# Autodesk Inventor assembly: Carril
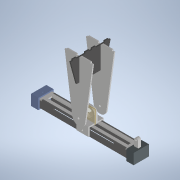
[picture p0: Inventor's stored thumbnail of the model, 180x180]
Saved by Autodesk Inventor 2022 (Build 260153000, 153)
## iProperties
Created: 2022-01-30
Part Number: Carril
Document SubType Name: Assembly
Designer: katha
Author: katha
## Documents named in this file (8)
- C:\Users\katha\OneDrive\Escritorio\Mini_Proyecto_Diseno\Diseno_18012\Modelo_MPD\Carril.iam
- C:\Users\katha\OneDrive\Escritorio\Mini_Proyecto_Diseno\Diseno_18012\Modelo_MPD\Lateral_Carril.ipt
- C:\Users\katha\OneDrive\Escritorio\Mini_Proyecto_Diseno\Diseno_18012\Modelo_MPD\Base_Carril.ipt
- C:\Users\katha\OneDrive\Escritorio\Mini_Proyecto_Diseno\Diseno_18012\Modelo_MPD\Tope_Carril.ipt
- C:\Users\katha\OneDrive\Escritorio\Mini_Proyecto_Diseno\Diseno_18012\Modelo_MPD\Tope_Carril_derecho.ipt
- C:\Users\katha\OneDrive\Escritorio\Mini_Proyecto_Diseno\Diseno_18012\Modelo_MPD\Eje_Carril.ipt
- C:\Users\katha\OneDrive\Escritorio\Mini_Proyecto_Diseno\Diseno_18012\Modelo_MPD\Base.ipt
- C:\Users\katha\OneDrive\Escritorio\Mini_Proyecto_Diseno\Diseno_18012\Modelo_MPD\Base_Soporte.ipt
## Components (9 placed, 7 different names)
1. Lateral_Carril:1 — Flush:1, Flush:3, Mate:2, Mate:4, Mate:7, Mate:18
2. Lateral_Carril:2 — Flush:2, Flush:4, Mate:1, Mate:10
3. Base_Carril:1 — Flush:1, Flush:2, Flush:3, Flush:4, Mate:1, Mate:2, Mate:3, Mate:5, Mate:6, Mate:8, Mate:17
4. Tope_Carril:1 — Mate:3, Mate:4, Mate:5
5. Tope_Carril_derecho:1 — Mate:6, Mate:7, Mate:8, Flush:6
6. Eje_Carril:1 — Mate:10, Mate:11, Mate:14, Mate:17, Mate:18, Flush:6
7. Base:1 — Mate:11, Flush:5, Mate:12, Mate:13, Mate:14, Mate:15, Mate:16
8. Base:2 — Flush:5, Mate:12, Mate:13
9. Base_Soporte:1 — Mate:15, Mate:16
## Relationships (23: Mate 17, Flush 6)
- Flush:1: Lateral_Carril:1 ↔ Base_Carril:1
- Flush:2: Lateral_Carril:2 ↔ Base_Carril:1
- Flush:3: Lateral_Carril:1 ↔ Base_Carril:1
- Flush:4: Lateral_Carril:2 ↔ Base_Carril:1
- Mate:1: Lateral_Carril:2 ↔ Base_Carril:1
- Mate:2: Lateral_Carril:1 ↔ Base_Carril:1
- Mate:3 (0.3 mm): Base_Carril:1 ↔ Tope_Carril:1
- Mate:4: Lateral_Carril:1 ↔ Tope_Carril:1
- Mate:5: Base_Carril:1 ↔ Tope_Carril:1
- Mate:6 (0.3 mm): Base_Carril:1 ↔ Tope_Carril_derecho:1
- Mate:7: Lateral_Carril:1 ↔ Tope_Carril_derecho:1
- Mate:8: Base_Carril:1 ↔ Tope_Carril_derecho:1
- Mate:10 (0.3 mm): Lateral_Carril:2 ↔ Eje_Carril:1
- Mate:11: Eje_Carril:1 ↔ Base:1
- Flush:5: Base:1 ↔ Base:2
- Mate:12 (50 mm): Base:1 ↔ Base:2
- Mate:13: Base:1 ↔ Base:2
- Mate:14 (21.25 mm): Eje_Carril:1 ↔ Base:1
- Mate:15: Base:1 ↔ Base_Soporte:1
- Mate:16: Base:1 ↔ Base_Soporte:1
- Mate:17 (0.2 mm): Base_Carril:1 ↔ Eje_Carril:1
- Mate:18 (0.119 mm): Lateral_Carril:1 ↔ Eje_Carril:1
- Flush:6: Tope_Carril_derecho:1 ↔ Eje_Carril:1
